# Autodesk Inventor assembly: Ensamble actuador faja
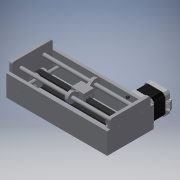
[picture p0: Inventor's stored thumbnail of the model, 180x180]
Saved by Autodesk Inventor 2019 (Build 230136000, 136)
## iProperties
Created: 2020-02-05
Part Number: Ensamble actuador faja
Document SubType Name: Assembly
Designer: Elías Sánchez
Author: Elías Sánchez
## Documents named in this file (17)
- D:\Documents\UVG\9no SEMESTRE\DISEÑO E INNOVACIÓN\Proyecto Actuadores\Inventor Actuadores\Actuador faja\Ensamble actuador faja.iam
- D:\Documents\UVG\9no SEMESTRE\DISEÑO E INNOVACIÓN\Proyecto Actuadores\Inventor Actuadores\Actuador faja\Nema 17\Nema_17-17HS4401.iam
- D:\Documents\UVG\9no SEMESTRE\DISEÑO E INNOVACIÓN\Proyecto Actuadores\Inventor Actuadores\Actuador faja\Acople eje motor.ipt
- D:\Documents\UVG\9no SEMESTRE\DISEÑO E INNOVACIÓN\Proyecto Actuadores\Inventor Actuadores\Actuador faja\Faja motor.ipt
- D:\Documents\UVG\9no SEMESTRE\DISEÑO E INNOVACIÓN\Proyecto Actuadores\Inventor Actuadores\Actuador faja\Riel.ipt
- D:\Documents\UVG\9no SEMESTRE\DISEÑO E INNOVACIÓN\Proyecto Actuadores\Inventor Actuadores\Actuador faja\Salida.ipt
- D:\Documents\UVG\9no SEMESTRE\DISEÑO E INNOVACIÓN\Proyecto Actuadores\Inventor Actuadores\Actuador faja\Tope riel final.ipt
- D:\Documents\UVG\9no SEMESTRE\DISEÑO E INNOVACIÓN\Proyecto Actuadores\Inventor Actuadores\Actuador faja\Tope riel motor 2.ipt
- D:\Documents\UVG\9no SEMESTRE\DISEÑO E INNOVACIÓN\Proyecto Actuadores\Inventor Actuadores\Actuador faja\Tope riel motor.ipt
- D:\Documents\UVG\9no SEMESTRE\DISEÑO E INNOVACIÓN\Proyecto Actuadores\Inventor Actuadores\Actuador faja\Anillo riel.ipt
- D:\Documents\UVG\9no SEMESTRE\DISEÑO E INNOVACIÓN\Proyecto Actuadores\Inventor Actuadores\Actuador faja\Faja motor largo.ipt
- D:\Documents\UVG\9no SEMESTRE\DISEÑO E INNOVACIÓN\Proyecto Actuadores\Inventor Actuadores\Actuador faja\Eje.ipt
- D:\Documents\UVG\9no SEMESTRE\DISEÑO E INNOVACIÓN\Proyecto Actuadores\Inventor Actuadores\Actuador faja\Eje 2.ipt
- D:\Documents\UVG\9no SEMESTRE\DISEÑO E INNOVACIÓN\Proyecto Actuadores\Inventor Actuadores\Actuador faja\M3.5.ipt
- D:\Documents\UVG\9no SEMESTRE\DISEÑO E INNOVACIÓN\Proyecto Actuadores\Inventor Actuadores\Actuador faja\M3.ipt
- D:\Documents\UVG\9no SEMESTRE\DISEÑO E INNOVACIÓN\Proyecto Actuadores\Inventor Actuadores\Actuador faja\faja.ipt
- D:\Documents\UVG\9no SEMESTRE\DISEÑO E INNOVACIÓN\Proyecto Actuadores\Inventor Actuadores\Actuador faja\Pin.ipt
## Components (23 placed, 16 different names)
1. Nema_17-17HS4401:1 [sub-assembly] — Mate:1, Insert:2, Insert:4
2. Acople eje motor:1 — Insert:2, Mate:18, Mate:19, Insert:13
3. Faja motor:1 — Mate:20, Mate:21, Mate:24, Mate:25
4. Riel:1 — Insert:6, Mate:14
5. Riel:2 — Insert:5
6. Salida:1 — Mate:8, Mate:9, Mate:10, Mate:11, Mate:12, Mate:13, Angle:2, Insert:14, Insert:15
7. Tope riel final:1 — Mate:6, Insert:5, Insert:6, Flush:3, Flush:4, Angle:2, Flush:5, Flush:6
8. Tope riel final:2 — Mate:3, Flush:1, Flush:2
9. Tope riel motor 2:1 — Mate:21, Mate:22, Flush:5, Flush:6, Insert:8
10. Anillo riel:1 — Mate:10, Mate:11, Mate:12
11. Anillo riel:2 — Mate:8, Mate:9, Mate:13, Mate:14
12. Tope riel motor:1 — Insert:4, Mate:4, Flush:1, Flush:2, Flush:3, Flush:4, Insert:7, Insert:9, Insert:10, Insert:11, Insert:12
13. Faja motor largo:1 — Mate:18, Mate:19
14. Eje:1 — Insert:7, Mate:20
15. Eje 2:1 — Insert:8, Mate:23
16. M3.5:1 — Insert:9
17. M3.5:2 — Insert:10
18. M3.5:3 — Insert:12
19. M3.5:4 — Insert:11
20. M3:1 — Insert:13
21. faja:1 — Mate:23, Mate:24, Mate:25
22. Pin:1 — Insert:14
23. Pin:2 — Insert:15
## Relationships (39: Mate 19, Insert 13, Flush 6, Angle 1)
- Mate:1: Nema_17-17HS4401:1
- Insert:2: Nema_17-17HS4401:1 ↔ Acople eje motor:1
- Mate:3: Tope riel final:2
- Insert:4 (-2 mm): Nema_17-17HS4401:1 ↔ Tope riel motor:1
- Mate:4: Tope riel motor:1
- Flush:1: Tope riel final:2 ↔ Tope riel motor:1
- Flush:2: Tope riel final:2 ↔ Tope riel motor:1
- Mate:6: Tope riel final:1
- Insert:5: Riel:2 ↔ Tope riel final:1
- Insert:6: Riel:1 ↔ Tope riel final:1
- Mate:8 (-10 mm): Salida:1 ↔ Anillo riel:2
- Mate:9: Salida:1 ↔ Anillo riel:2
- Mate:10 (-10 mm): Salida:1 ↔ Anillo riel:1
- Mate:11: Salida:1 ↔ Anillo riel:1
- Mate:12: Salida:1 ↔ Anillo riel:1
- Mate:13: Salida:1 ↔ Anillo riel:2
- Mate:14: Riel:1 ↔ Anillo riel:2
- Flush:3: Tope riel final:1 ↔ Tope riel motor:1
- Flush:4: Tope riel final:1 ↔ Tope riel motor:1
- Angle:2 (0 deg): Salida:1 ↔ Tope riel final:1
- Mate:18: Acople eje motor:1 ↔ Faja motor largo:1
- Mate:19: Acople eje motor:1 ↔ Faja motor largo:1
- Insert:7 (-6 mm): Tope riel motor:1 ↔ Eje:1
- Mate:20: Faja motor:1 ↔ Eje:1
- Mate:21 (30 mm): Faja motor:1 ↔ Tope riel motor 2:1
- Mate:22: Tope riel motor 2:1
- Flush:5: Tope riel final:1 ↔ Tope riel motor 2:1
- Flush:6: Tope riel final:1 ↔ Tope riel motor 2:1
- Insert:8: Tope riel motor 2:1 ↔ Eje 2:1
- Insert:9: Tope riel motor:1 ↔ M3.5:1
- Insert:10: Tope riel motor:1 ↔ M3.5:2
- Insert:11: Tope riel motor:1 ↔ M3.5:4
- Insert:12: Tope riel motor:1 ↔ M3.5:3
- Insert:13: Acople eje motor:1 ↔ M3:1
- Mate:23: Eje 2:1 ↔ faja:1
- Mate:24 (1 mm): Faja motor:1 ↔ faja:1
- Mate:25: Faja motor:1 ↔ faja:1
- Insert:14: Salida:1 ↔ Pin:1
- Insert:15: Salida:1 ↔ Pin:2
